# Autodesk Inventor assembly: set2_to_print_modified
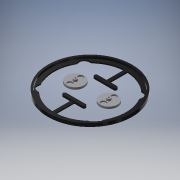
[picture p0: Inventor's stored thumbnail of the model, 180x180]
Saved by Autodesk Inventor 2017 SP1 (Build 210196100, 196)
## iProperties
Created: 2016-07-26
Part Number: set2_to_print_modified
Material: Générique
Document SubType Name: Assembly
Designer: tmonglon
Author: tmonglon
## Documents named in this file (3)
- D:\Inventor\Ahmet\29_mai_2017\20170525_ebug_chassis\modified\set2_to_print_modified.iam
- D:\Inventor\Ahmet\magnet_holder.ipt
- D:\Inventor\Ahmet\mai_2017\modified\bumper_modified2.ipt
## Components (3 placed, 2 different names)
1. magnet_holder:1 — Placage:3, Angle:1, Affleurement:1, Placage:6
2. magnet_holder:2 — Placage:4, Angle:2, Affleurement:1, Placage:7
3. bumper_modified2:1 — Placage:1, Placage:2, Angle:1, Angle:2, Placage:5
## Relationships (10: Mate 7, Angle 2, Flush 1)
- Placage:1 [Mate]: bumper_modified2:1
- Placage:2 [Mate]: bumper_modified2:1
- Placage:3 [Mate]: magnet_holder:1
- Placage:4 [Mate]: magnet_holder:2
- Angle:1 (90 deg): magnet_holder:1 ↔ bumper_modified2:1
- Angle:2 (90 deg): magnet_holder:2 ↔ bumper_modified2:1
- Placage:5 [Mate]: bumper_modified2:1
- Affleurement:1 [Flush]: magnet_holder:1 ↔ magnet_holder:2
- Placage:6 [Mate]: magnet_holder:1
- Placage:7 [Mate]: magnet_holder:2
